# Autodesk Inventor assembly: Hand Assembly
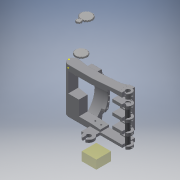
[picture p0: Inventor's stored thumbnail of the model, 180x180]
Saved by Autodesk Inventor 2017 (Build 210142000, 142)
## iProperties
Created: 2016-09-28
Part Number: Hand Assembly
Document SubType Name: Assembly
Designer: cmcdona
Author: cmcdona
## Documents named in this file (14)
- D:\julie\Documents\Cours McMaster\Graphics & Design\Project\Hand Assembly.iam
- D:\julie\Documents\Cours McMaster\Graphics & Design\Project\Hand - Frame.ipt
- D:\julie\Documents\Cours McMaster\Graphics & Design\Project\Hand - Digit 4.ipt
- D:\julie\Documents\Cours McMaster\Graphics & Design\Project\Hand - Digit 0-1.ipt
- D:\julie\Documents\Cours McMaster\Graphics & Design\Project\Hand - Distal Bridge.ipt
- D:\julie\Documents\Cours McMaster\Graphics & Design\Project\Hand - Digit 2-3.ipt
- D:\julie\Documents\Cours McMaster\Graphics & Design\Project\Hand - Proximal Bridge.ipt
- D:\julie\Documents\Cours McMaster\Graphics & Design\Project\Hand - Functional Workspace.ipt
- D:\julie\Documents\Cours McMaster\Graphics & Design\Project\Input Motor.ipt
- D:\julie\Documents\Cours McMaster\Graphics & Design\Project\Hand Assembly\Design Accelerator\Spur Gears1.iam
- D:\julie\Documents\Cours McMaster\Graphics & Design\Project\Hand Assembly\Design Accelerator\Spur Gears2.iam
- D:\julie\Documents\Cours McMaster\Graphics & Design\Project\Forefingers Rod.ipt
- D:\julie\Documents\Cours McMaster\Graphics & Design\Project\Hand Assembly\Design Accelerator\Spur Gear11.ipt
- D:\julie\Documents\Cours McMaster\Graphics & Design\Project\Hand Assembly\Design Accelerator\Spur Gear21.ipt
## Components (15 placed, 12 different names)
1. Hand - Frame:1 — Flush:1, Flush:2, Mate:1, Mate:2, Flush:3, Mate:3, Mate:16, Mate:17, Mate:18, Mate:22, Mate:23
2. Hand - Digit 4:1 — Flush:1, Flush:2, Mate:1, Mate:4, Mate:5, Mate:24
3. Hand - Digit 0-1:1 — Mate:2, Flush:3, Mate:3, Mate:6, Mate:19, Mate:20, Mate:21, Flush:4
4. Hand - Distal Bridge:1 — Mate:4, Mate:5, Mate:6, Mate:7, Mate:8, Mate:9, Mate:10, Mate:11, Mate:12, Mate:13, Mate:14, Mate:15
5. Hand - Digit 2-3:1 — Mate:7, Mate:8, Mate:9
6. Hand - Digit 2-3:2 — Mate:10, Mate:11, Mate:12
7. Hand - Digit 2-3:3 — Mate:13, Mate:14, Mate:15
8. Hand - Proximal Bridge:1 — Mate:16, Mate:17, Mate:18
9. Hand - Functional Workspace:1 — Mate:19, Mate:20, Mate:21
10. Input Motor:1 — Mate:22, Mate:23, Mate:25
11. Spur Gears:1 [sub-assembly]
12. Spur Gears:2 [sub-assembly]
13. Forefingers Rod:1 — Mate:24, Flush:4
14. Spur Gear1:1 — Mate:25
15. Spur Gear2:1
## Relationships (29: Mate 25, Flush 4)
- Flush:1: Hand - Frame:1 ↔ Hand - Digit 4:1
- Flush:2: Hand - Frame:1 ↔ Hand - Digit 4:1
- Mate:1: Hand - Frame:1 ↔ Hand - Digit 4:1
- Mate:2: Hand - Frame:1 ↔ Hand - Digit 0-1:1
- Flush:3: Hand - Frame:1 ↔ Hand - Digit 0-1:1
- Mate:3: Hand - Frame:1 ↔ Hand - Digit 0-1:1
- Mate:4: Hand - Digit 4:1 ↔ Hand - Distal Bridge:1
- Mate:5: Hand - Digit 4:1 ↔ Hand - Distal Bridge:1
- Mate:6: Hand - Digit 0-1:1 ↔ Hand - Distal Bridge:1
- Mate:7: Hand - Distal Bridge:1 ↔ Hand - Digit 2-3:1
- Mate:8: Hand - Distal Bridge:1 ↔ Hand - Digit 2-3:1
- Mate:9: Hand - Distal Bridge:1 ↔ Hand - Digit 2-3:1
- Mate:10: Hand - Distal Bridge:1 ↔ Hand - Digit 2-3:2
- Mate:11: Hand - Distal Bridge:1 ↔ Hand - Digit 2-3:2
- Mate:12: Hand - Distal Bridge:1 ↔ Hand - Digit 2-3:2
- Mate:13: Hand - Distal Bridge:1 ↔ Hand - Digit 2-3:3
- Mate:14: Hand - Distal Bridge:1 ↔ Hand - Digit 2-3:3
- Mate:15: Hand - Distal Bridge:1 ↔ Hand - Digit 2-3:3
- Mate:16: Hand - Frame:1 ↔ Hand - Proximal Bridge:1
- Mate:17: Hand - Frame:1 ↔ Hand - Proximal Bridge:1
- Mate:18: Hand - Frame:1 ↔ Hand - Proximal Bridge:1
- Mate:19: Hand - Digit 0-1:1 ↔ Hand - Functional Workspace:1
- Mate:20 (41 mm): Hand - Digit 0-1:1 ↔ Hand - Functional Workspace:1
- Mate:21 (33 mm): Hand - Digit 0-1:1 ↔ Hand - Functional Workspace:1
- Mate:22: Hand - Frame:1 ↔ Input Motor:1
- Mate:23: Hand - Frame:1 ↔ Input Motor:1
- Mate:24: Hand - Digit 4:1 ↔ Forefingers Rod:1
- Flush:4: Hand - Digit 0-1:1 ↔ Forefingers Rod:1
- Mate:25: Input Motor:1 ↔ Spur Gear1:1
